# Autodesk Inventor assembly: CIM Key Shaft Connecter
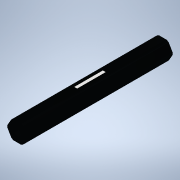
[picture p0: Inventor's stored thumbnail of the model, 180x180]
Saved by Autodesk Inventor 2020 (Build 240168000, 168)
## iProperties
Created: 2020-02-02
Part Number: CIM Key Shaft Connecter
Document SubType Name: Assembly
Designer: aidan
Author: aidan
## Documents named in this file (3)
- C:\Users\aidan\Desktop\T3 Robotics\CAD\CIM Key Shaft Connecter.iam
- C:\Users\aidan\Desktop\T3 Robotics\CAD\Thundershaft 2in.ipt
- C:\Users\aidan\Desktop\T3 Robotics\CAD\Maybe CIM Key.ipt
## Components (3 placed, 2 different names)
1. Thundershaft 2in:1 — Mate:1, Flush:1, Flush:2, Mate:2, Mate:3, Flush:3
2. Thundershaft 2in:2 — Mate:1, Flush:1, Flush:2
3. Maybe CIM Key:1 — Mate:2, Mate:3, Flush:3
## Relationships (6: Mate 3, Flush 3)
- Mate:1: Thundershaft 2in:1 ↔ Thundershaft 2in:2
- Flush:1: Thundershaft 2in:1 ↔ Thundershaft 2in:2
- Flush:2: Thundershaft 2in:1 ↔ Thundershaft 2in:2
- Mate:2: Thundershaft 2in:1 ↔ Maybe CIM Key:1
- Mate:3: Thundershaft 2in:1 ↔ Maybe CIM Key:1
- Flush:3: Thundershaft 2in:1 ↔ Maybe CIM Key:1
